# Autodesk Inventor assembly: FullField-ver1-1111-2021
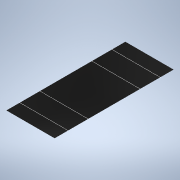
[picture p0: Inventor's stored thumbnail of the model, 180x180]
Saved by Autodesk Inventor 2021 (Build 250183000, 183)
## iProperties
Created: 2021-02-23
Part Number: FullField-ver1-1111-2021
Document SubType Name: Assembly
Designer: CMurray
Author: CMurray
## Documents named in this file (3)
- F:\PHRC CADD 2021\2021 Game Design Challenge\Full Field\FullField-ver1-1111-2021.iam
- F:\PH Robotics 2020 Field CAD\Parts\FE-2020-01.ipt
- F:\PHRC CADD 2021\2021 Game Design Challenge\Tape\Tape.ipt
## Components (6 placed, 2 different names)
1. FE-2020-01:1 — Mate:1, Flush:1, Flush:2, Mate:3, Flush:3, Flush:4, Flush:5, Flush:6, Mate:4, Flush:7, Flush:8
2. FE-2020-01:2 — Mate:1, Flush:1, Mate:2, Flush:3, Mate:6
3. Tape:1 — Mate:2, Flush:2, Flush:5, Mate:5
4. Tape:2 — Mate:3, Flush:4, Flush:6, Mate:7
5. Tape:3 — Mate:4, Flush:7, Mate:5
6. Tape:4 — Mate:6, Flush:8, Mate:7
## Relationships (15: Flush 8, Mate 7)
- Mate:1: FE-2020-01:1 ↔ FE-2020-01:2
- Flush:1: FE-2020-01:1 ↔ FE-2020-01:2
- Mate:2: FE-2020-01:2 ↔ Tape:1
- Flush:2: FE-2020-01:1 ↔ Tape:1
- Mate:3: FE-2020-01:1 ↔ Tape:2
- Flush:3: FE-2020-01:1 ↔ FE-2020-01:2
- Flush:4: FE-2020-01:1 ↔ Tape:2
- Flush:5 (2514.6 mm): FE-2020-01:1 ↔ Tape:1
- Flush:6 (2514.6 mm): FE-2020-01:1 ↔ Tape:2
- Mate:4: FE-2020-01:1 ↔ Tape:3
- Flush:7: FE-2020-01:1 ↔ Tape:3
- Mate:5 (3759.2 mm): Tape:1 ↔ Tape:3
- Mate:6: FE-2020-01:2 ↔ Tape:4
- Flush:8: FE-2020-01:1 ↔ Tape:4
- Mate:7 (3759.2 mm): Tape:2 ↔ Tape:4
